# Autodesk Inventor assembly: Drill JIg Assembly v3
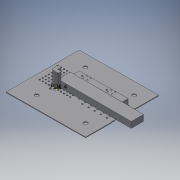
[picture p0: Inventor's stored thumbnail of the model, 180x180]
Saved by Autodesk Inventor 2018 (Build 220112000, 112)
## iProperties
Created: 2018-12-13
Part Number: Drill JIg Assembly v3
Document SubType Name: Assembly
Designer: Gabriel
Author: Gabriel
## Documents named in this file (5)
- C:\Users\Gabriel\Documents\GitHub\2019CAD\Drill Jig Files\Drill JIg Assembly v3.iam
- C:\Users\Gabriel\Documents\GitHub\2019CAD\Drill Jig Files\Drill Jig Base 2.ipt
- C:\Users\Gabriel\Documents\GitHub\2019CAD\Drill Jig Files\Clamp Mount Aligner.ipt
- C:\Users\Gabriel\Documents\GitHub\2019CAD\Drill Jig Files\Jig2.1_1x1_Bolt_Pattern_PIN.ipt
- C:\Users\Gabriel\Documents\GitHub\2019CAD\Drill Jig Files\1x2 Beam Test.ipt
## Components (4 placed, 4 different names)
1. Drill Jig Base 2:1 — Mate:1, Mate:2, Mate:3, Mate:4
2. Clamp Mount Aligner:1 — Mate:1, Mate:2
3. Jig2.1_1x1_Bolt_Pattern_PIN:1 — Mate:3, Mate:4
4. 1x2 Beam Test:1
## Relationships (4: Mate 4)
- Mate:1: Drill Jig Base 2:1 ↔ Clamp Mount Aligner:1
- Mate:2: Drill Jig Base 2:1 ↔ Clamp Mount Aligner:1
- Mate:3: Drill Jig Base 2:1 ↔ Jig2.1_1x1_Bolt_Pattern_PIN:1
- Mate:4: Drill Jig Base 2:1 ↔ Jig2.1_1x1_Bolt_Pattern_PIN:1
